# Autodesk Inventor assembly: Assembly1
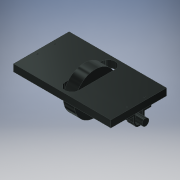
[picture p0: Inventor's stored thumbnail of the model, 180x180]
Saved by Autodesk Inventor 2018 (Build 220112000, 112)
## iProperties
Created: 2021-03-01
Part Number: Assembly1
Document SubType Name: Assembly
Designer: Default
Author: Default
## Documents named in this file (7)
- F:\AUTODESK PROJECTS\Assembly1.iam
- F:\AUTODESK PROJECTS\disk plate.ipt
- F:\AUTODESK PROJECTS\2wheel.ipt
- F:\AUTODESK PROJECTS\shaft.ipt
- F:\AUTODESK PROJECTS\Assembly1\Design Accelerator\Bearing3.iam
- F:\AUTODESK PROJECTS\saddle 3.ipt
- F:\AUTODESK PROJECTS\Assembly1\Design Accelerator\Bolted Connection1.iam
## Components (7 placed, 6 different names)
1. disk plate:1 — Mate:2, Mate:4, Mate:5, Mate:6, Mate:7
2. 2wheel:1 — Flush:1, Mate:2, Mate:3
3. shaft:1 — Mate:1, Flush:1, Mate:3
4. Bearing:1 [sub-assembly] — Mate:1
5. saddle 3:1 — Mate:4, Mate:5
6. saddle 3:2 — Mate:6, Mate:7, Mate:8, Mate:9
7. Bolted Connection:1 [sub-assembly] — Mate:8, Mate:9
## Relationships (10: Mate 9, Flush 1)
- Mate:1: shaft:1 ↔ Bearing:1
- Flush:1 (180 mm): 2wheel:1 ↔ shaft:1
- Mate:2 (5 mm): disk plate:1 ↔ 2wheel:1
- Mate:3: 2wheel:1 ↔ shaft:1
- Mate:4: disk plate:1 ↔ saddle 3:1
- Mate:5: disk plate:1 ↔ saddle 3:1
- Mate:6: disk plate:1 ↔ saddle 3:2
- Mate:7: disk plate:1 ↔ saddle 3:2
- Mate:8: saddle 3:2 ↔ Bolted Connection:1
- Mate:9: saddle 3:2 ↔ Bolted Connection:1
